# Autodesk Inventor assembly: hatch above arm
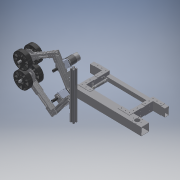
[picture p0: Inventor's stored thumbnail of the model, 180x180]
Saved by Autodesk Inventor 2018 (Build 220112000, 112)
## iProperties
Created: 2019-01-20
Part Number: hatch above arm
Document SubType Name: Assembly
Designer: Burni
Author: Burni
## Documents named in this file (3)
- C:\Users\s-4008082\Downloads\2019CAD-master\2019CAD-master\new Hatch design but everythig is broke\hatch above arm.iam
- C:\Users\s-4008082\Downloads\2019CAD-master  DELETE OTHERS(4)\2019CAD-master\Ball Intake ver 2\MAIN Gripper assembly.iam
- C:\Users\s-4008082\Downloads\2019CAD-master\2019CAD-master\new Hatch design but everythig is broke\non integrated hatch.iam
## Components (2 placed, 2 different names)
1. MAIN Gripper assembly:1 [sub-assembly] — Mate:1
2. non integrated hatch:1 [sub-assembly] — Mate:1
## Relationships (1: Mate 1)
- Mate:1: MAIN Gripper assembly:1 ↔ non integrated hatch:1
